# Autodesk Inventor assembly: Box
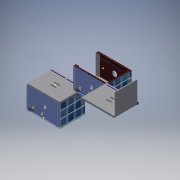
[picture p0: Inventor's stored thumbnail of the model, 180x180]
Saved by Autodesk Inventor 2018 (Build 220112000, 112)
## iProperties
Created: 2018-04-07
Part Number: Box
Document SubType Name: Assembly
Designer: MIABo
Author: MIABo
## Documents named in this file (3)
- C:\Users\MIABo\Documents\GitHub\Ares1\3D Model Files\Box.iam
- C:\Users\MIABo\Documents\GitHub\Ares1\3D Model Files\Boxpt1.ipt
- C:\Users\MIABo\Documents\GitHub\Ares1\3D Model Files\Boxpt2.ipt
## Components (4 placed, 2 different names)
1. Boxpt1:1 — Mate:1, Mate:2, Mate:3
2. Boxpt2:1 — Mate:1, Mate:2, Mate:3
3. Boxpt1:2
4. Boxpt2:2
## Relationships (3: Mate 3)
- Mate:1: Boxpt1:1 ↔ Boxpt2:1
- Mate:2: Boxpt1:1 ↔ Boxpt2:1
- Mate:3: Boxpt1:1 ↔ Boxpt2:1
